# Autodesk Inventor assembly: A2_PongBoy
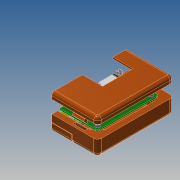
[picture p0: Inventor's stored thumbnail of the model, 180x180]
Saved by Autodesk Inventor 2020.2 (Build 242310000, 310)
## iProperties
Created: 2021-08-30
Part Number: A2_PongBoy
Document SubType Name: Assembly
Designer: Samy Francelet
Author: Samy Francelet
## Documents named in this file (5)
- D:\work\PongBoy\0400_Mechanical\A2_PongBoy.iam
- D:\work\PongBoy\0400_Mechanical\P1_BottomCase.ipt
- D:\work\PongBoy\0400_Mechanical\A1_PCB.iam
- D:\work\PongBoy\0400_Mechanical\P3_BatteriesTray.ipt
- D:\work\PongBoy\0400_Mechanical\P2_TopCase.ipt
## Components (4 placed, 4 different names)
1. P1_BottomCase:1 — Placage:1, Placage:2, Placage:3, Placage:4, Placage:5, Affleurement:1, Placage:6, Affleurement:2
2. A1_PCB:1 [sub-assembly] — Placage:1, Placage:2, Placage:3
3. P3_BatteriesTray:1 — Placage:4, Placage:5, Affleurement:1
4. P2_TopCase:1 — Placage:6, Affleurement:2
## Relationships (8: Mate 6, Flush 2)
- Placage:1 [Mate]: P1_BottomCase:1 ↔ A1_PCB:1
- Placage:2 [Mate]: P1_BottomCase:1 ↔ A1_PCB:1
- Placage:3 [Mate]: P1_BottomCase:1 ↔ A1_PCB:1
- Placage:4 [Mate]: P1_BottomCase:1 ↔ P3_BatteriesTray:1
- Placage:5 [Mate]: P1_BottomCase:1 ↔ P3_BatteriesTray:1
- Affleurement:1 [Flush]: P1_BottomCase:1 ↔ P3_BatteriesTray:1
- Placage:6 [Mate] (0.5 mm): P1_BottomCase:1 ↔ P2_TopCase:1
- Affleurement:2 [Flush]: P1_BottomCase:1 ↔ P2_TopCase:1
